# Autodesk Inventor assembly: GripperV2
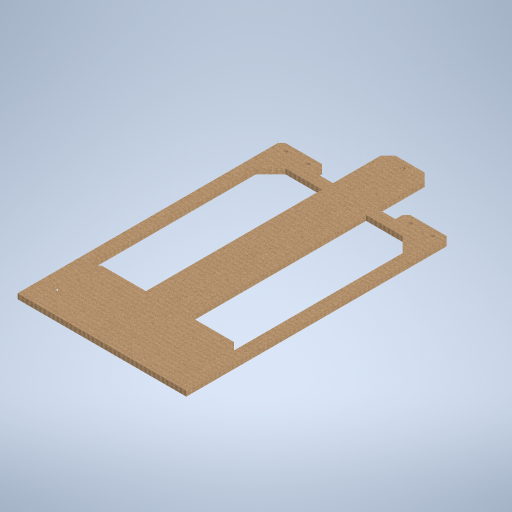
[picture p0: Inventor's stored thumbnail of the model, 512x512]
Saved by Autodesk Inventor 2023.1 (Build 271208000, 208)
## iProperties
Created: 2022-10-30
Part Number: GripperV2
Document SubType Name: Assembly
Designer: Daniel Peña
Author: Daniel Peña
## Documents named in this file (3)
- E:\Daniel DiscoA\Documents\UNAL\ProyectoRobotica\CAD\GripperV2.iam
- E:\Daniel DiscoA\Documents\UNAL\ProyectoRobotica\CAD\MarcoV2.ipt
- E:\Daniel DiscoA\Documents\UNAL\ProyectoRobotica\CAD\PistonV2.ipt
## Components (2 placed, 2 different names)
1. MarcoV2:1 — Piston
2. PistonV2:1 — Piston
## Relationships (1: TranslationJoint 1)
- Piston [TranslationJoint]: MarcoV2:1 ↔ PistonV2:1
